# Autodesk Inventor assembly: 2009_CTS_SpeedController
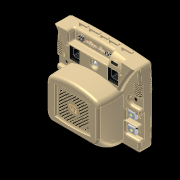
[picture p0: Inventor's stored thumbnail of the model, 180x180]
Saved by Autodesk Inventor 2012 (Build 160160000, 160)
## iProperties
Company: Team 801
Created: 2009-01-31
Part Number: 2009_CTS_SpeedController
Document SubType Name: Assembly
Designer: Jeffrey M
Description: Fully Assembled Jagaur
Mass: 2133.46 g
Surface Area: 664.309 cm^2
Volume: 301.606 cm^3
Density: 7.07366 g/cm^3
Title: 2009_CTS_SpeedController
Author: Jeffrey M
## Documents named in this file (7)
- Z:\UserData\Documents\Inventor\team1885frc\Electronics\Jag\Jag.iam
- Z:\UserData\Documents\Inventor\team1885frc\Electronics\Jag\BasicShape.ipt
- Z:\UserData\Documents\Inventor\team1885frc\Electronics\Jag\UClip.ipt
- Z:\UserData\Documents\Inventor\team1885frc\Electronics\Jag\Light.ipt
- Z:\UserData\Documents\Inventor\team1885frc\Electronics\Jag\CopperPost.ipt
- Z:\UserData\Documents\Inventor\team1885frc\Electronics\Jag\EatherNetPort.ipt
- Z:\UserData\Documents\Inventor\team1885frc\Electronics\Jag\CopperPost2.ipt
## Components (20 placed, 6 different names)
1. BasicShape:1 — Angle:1, Angle:2, Mate:1, Mate:2, Mate:3, Mate:4, Mate:5, Mate:6, Mate:7, Mate:8, Mate:9, Mate:10, Mate:11, Mate:12, Mate:13, Angle:11, Angle:12, Mate:14, Mate:15, Mate:16, Angle:13, Angle:14, Mate:17, Mate:18, Mate:19, Mate:21, Mate:22, Mate:23, Mate:24, Angle:20, Mate:26, Mate:27, Mate:28, Mate:29, Mate:31, Mate:32, Mate:34, Mate:35, Mate:37, Mate:38, Mate:39, Angle:31, Angle:32, Mate:41, Mate:42, Mate:43, Angle:33, Angle:34, Mate:44, Mate:45, Mate:46, Angle:35, Angle:36, Mate:47, Mate:48, Mate:49, Angle:37, Mate:50, Mate:51, Mate:52, Mate:53, Mate:54
2. UClip:1 — Angle:1, Angle:2, Mate:1, Mate:2, Mate:3, Angle:3, Angle:4, Angle:5, Angle:6
3. UClip:2 — Angle:3, Angle:4, Mate:4, Mate:5, Mate:6
4. UClip:3 — Angle:7, Angle:8, Mate:7, Mate:11, Mate:12
5. UClip:4 — Angle:5, Angle:6, Angle:7, Angle:8, Mate:8, Mate:9, Mate:10
6. Light:1 — Mate:13, Angle:9, Angle:10
7. CopperPost:1 — Angle:11, Angle:12, Mate:14, Mate:15, Mate:16, Angle:19
8. CopperPost:2 — Angle:15, Angle:16, Mate:20, Mate:21, Mate:22, Mate:25
9. CopperPost:3 — Angle:17, Angle:18, Mate:23, Mate:24, Mate:25
10. CopperPost:4 — Angle:13, Angle:14, Angle:15, Angle:16, Angle:17, Angle:18, Mate:17, Mate:18, Mate:19, Mate:20
11. CopperPost:5 — Angle:22, Angle:23, Angle:27, Angle:28, Mate:26, Mate:27, Mate:28, Mate:30, Angle:38
12. CopperPost:6 — Angle:21, Angle:26, Mate:32, Mate:33, Mate:34, Mate:36
13. CopperPost:7 — Angle:23, Angle:28, Mate:29, Mate:30, Mate:31, Mate:33
14. CopperPost:8 — Angle:19, Angle:20, Angle:21, Angle:22, Angle:24, Angle:25, Angle:26, Angle:27, Mate:35, Mate:36, Mate:37, Mate:40
15. CopperPost:9 — Angle:24, Angle:25, Mate:38, Mate:39, Mate:40
16. EatherNetPort:2 — Angle:31, Angle:32, Mate:41, Mate:42, Mate:43
17. EatherNetPort:3 — Angle:33, Angle:34, Mate:44, Mate:45, Mate:46
18. CopperPost2:1 — Angle:35, Angle:36, Mate:47, Mate:48, Mate:49
19. CopperPost2:2 — Angle:39, Angle:40, Mate:50, Mate:51, Mate:52, Mate:55
20. CopperPost2:3 — Angle:37, Angle:38, Angle:39, Angle:40, Mate:53, Mate:54, Mate:55
## Relationships (93: Mate 55, Angle 38)
- Angle:1 (0 deg): BasicShape:1 ↔ UClip:1
- Angle:2 (0 deg): BasicShape:1 ↔ UClip:1
- Mate:1: BasicShape:1 ↔ UClip:1
- Mate:2: BasicShape:1 ↔ UClip:1
- Mate:3: BasicShape:1 ↔ UClip:1
- Angle:3 (0 deg): UClip:1 ↔ UClip:2
- Angle:4 (0 deg): UClip:1 ↔ UClip:2
- Mate:4: BasicShape:1 ↔ UClip:2
- Mate:5: BasicShape:1 ↔ UClip:2
- Mate:6: BasicShape:1 ↔ UClip:2
- Angle:5 (0 deg): UClip:1 ↔ UClip:4
- Angle:6 (0 deg): UClip:1 ↔ UClip:4
- Angle:7 (0 deg): UClip:3 ↔ UClip:4
- Angle:8 (0 deg): UClip:3 ↔ UClip:4
- Mate:7: BasicShape:1 ↔ UClip:3
- Mate:8: BasicShape:1 ↔ UClip:4
- Mate:9: BasicShape:1 ↔ UClip:4
- Mate:10: BasicShape:1 ↔ UClip:4
- Mate:11: BasicShape:1 ↔ UClip:3
- Mate:12: BasicShape:1 ↔ UClip:3
- Mate:13: BasicShape:1 ↔ Light:1
- Angle:9 (0 deg): Light:1
- Angle:10 (0 deg): Light:1
- Angle:11 (0 deg): BasicShape:1 ↔ CopperPost:1
- Angle:12 (0 deg): BasicShape:1 ↔ CopperPost:1
- Mate:14: BasicShape:1 ↔ CopperPost:1
- Mate:15: BasicShape:1 ↔ CopperPost:1
- Mate:16: BasicShape:1 ↔ CopperPost:1
- Angle:13 (0 deg): BasicShape:1 ↔ CopperPost:4
- Angle:14 (0 deg): BasicShape:1 ↔ CopperPost:4
- Angle:15 (0 deg): CopperPost:2 ↔ CopperPost:4
- Angle:16 (0 deg): CopperPost:2 ↔ CopperPost:4
- Angle:17 (0 deg): CopperPost:3 ↔ CopperPost:4
- Angle:18 (0 deg): CopperPost:3 ↔ CopperPost:4
- Mate:17: BasicShape:1 ↔ CopperPost:4
- Mate:18: BasicShape:1 ↔ CopperPost:4
- Mate:19: BasicShape:1 ↔ CopperPost:4
- Mate:20: CopperPost:2 ↔ CopperPost:4
- Mate:21: BasicShape:1 ↔ CopperPost:2
- Mate:22: BasicShape:1 ↔ CopperPost:2
- Mate:23: BasicShape:1 ↔ CopperPost:3
- Mate:24: BasicShape:1 ↔ CopperPost:3
- Mate:25: CopperPost:2 ↔ CopperPost:3
- Angle:19 (0 deg): CopperPost:1 ↔ CopperPost:8
- Angle:20 (0 deg): BasicShape:1 ↔ CopperPost:8
- Angle:21 (0 deg): CopperPost:6 ↔ CopperPost:8
- Angle:22 (0 deg): CopperPost:5 ↔ CopperPost:8
- Angle:23 (0 deg): CopperPost:5 ↔ CopperPost:7
- Angle:24 (0 deg): CopperPost:8 ↔ CopperPost:9
- Angle:25 (0 deg): CopperPost:8 ↔ CopperPost:9
- Angle:26 (0 deg): CopperPost:6 ↔ CopperPost:8
- Angle:27 (0 deg): CopperPost:5 ↔ CopperPost:8
- Angle:28 (0 deg): CopperPost:5 ↔ CopperPost:7
- Mate:26: BasicShape:1 ↔ CopperPost:5
- Mate:27: BasicShape:1 ↔ CopperPost:5
- Mate:28 (-0.254 mm): BasicShape:1 ↔ CopperPost:5
- Mate:29: BasicShape:1 ↔ CopperPost:7
- Mate:30: CopperPost:5 ↔ CopperPost:7
- Mate:31: BasicShape:1 ↔ CopperPost:7
- Mate:32: BasicShape:1 ↔ CopperPost:6
- Mate:33: CopperPost:6 ↔ CopperPost:7
- Mate:34: BasicShape:1 ↔ CopperPost:6
- Mate:35: BasicShape:1 ↔ CopperPost:8
- Mate:36: CopperPost:6 ↔ CopperPost:8
- Mate:37: BasicShape:1 ↔ CopperPost:8
- Mate:38: BasicShape:1 ↔ CopperPost:9
- Mate:39: BasicShape:1 ↔ CopperPost:9
- Mate:40 (-0.508 mm): CopperPost:8 ↔ CopperPost:9
- Angle:31 (0 deg): BasicShape:1 ↔ EatherNetPort:2
- Angle:32 (0 deg): BasicShape:1 ↔ EatherNetPort:2
- Mate:41: BasicShape:1 ↔ EatherNetPort:2
- Mate:42: BasicShape:1 ↔ EatherNetPort:2
- Mate:43: BasicShape:1 ↔ EatherNetPort:2
- Angle:33 (0 deg): BasicShape:1 ↔ EatherNetPort:3
- Angle:34 (0 deg): BasicShape:1 ↔ EatherNetPort:3
- Mate:44: BasicShape:1 ↔ EatherNetPort:3
- Mate:45: BasicShape:1 ↔ EatherNetPort:3
- Mate:46: BasicShape:1 ↔ EatherNetPort:3
- Angle:35 (0 deg): BasicShape:1 ↔ CopperPost2:1
- Angle:36 (0 deg): BasicShape:1 ↔ CopperPost2:1
- Mate:47: BasicShape:1 ↔ CopperPost2:1
- Mate:48: BasicShape:1 ↔ CopperPost2:1
- Mate:49: BasicShape:1 ↔ CopperPost2:1
- Angle:37 (0 deg): BasicShape:1 ↔ CopperPost2:3
- Angle:38 (0 deg): CopperPost:5 ↔ CopperPost2:3
- Angle:39 (0 deg): CopperPost2:2 ↔ CopperPost2:3
- Angle:40 (0 deg): CopperPost2:2 ↔ CopperPost2:3
- Mate:50: BasicShape:1 ↔ CopperPost2:2
- Mate:51 (0.254 mm): BasicShape:1 ↔ CopperPost2:2
- Mate:52 (0.254 mm): BasicShape:1 ↔ CopperPost2:2
- Mate:53: BasicShape:1 ↔ CopperPost2:3
- Mate:54 (0.254 mm): BasicShape:1 ↔ CopperPost2:3
- Mate:55: CopperPost2:2 ↔ CopperPost2:3
